# Autodesk Inventor assembly: Frame
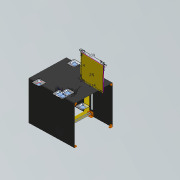
[picture p0: Inventor's stored thumbnail of the model, 180x180]
Saved by Autodesk Inventor 2016 (Build 200138000, 138)
## iProperties
Created: 2016-08-20
Part Number: Frame
Document SubType Name: Assembly
Designer: Sam
Author: Sam
## Documents named in this file (22)
- D:\Users\Sam\Documents\Inventor\Zircon3D\Frame.iam
- D:\Users\Sam\Documents\Inventor\Zircon3D\FrameBase.ipt
- D:\Users\Sam\Documents\Inventor\Zircon3D\FrameCentre.ipt
- D:\Users\Sam\Documents\Inventor\Zircon3D\FrameBack.ipt
- D:\Users\Sam\Documents\Inventor\Zircon3D\Frame3WayBlock.ipt
- D:\Users\Sam\Documents\Inventor\Zircon3D\FrameLeftSide.ipt
- D:\Users\Sam\Documents\Inventor\Zircon3D\FrameTop.ipt
- D:\Users\Sam\Documents\Inventor\Zircon3D\Frame2WayBlock.ipt
- D:\Users\Sam\Documents\Inventor\Zircon3D\FrameRightSide.ipt
- D:\Users\Sam\Documents\Inventor\Zircon3D\Frame Front.ipt
- D:\Users\Sam\Documents\Inventor\Zircon3D\Frame3WayBlockMotor.ipt
- D:\Users\Sam\Documents\Inventor\Zircon3D\SmoothRods.ipt
- D:\Users\Sam\Documents\Inventor\Zircon3D\MotorMountRight.ipt
- D:\Users\Sam\Documents\Inventor\Zircon3D\Frame3WayBlockMotor_MIR.ipt
- D:\Users\Sam\Documents\Inventor\Zircon3D\Nema17.ipt
- D:\Users\Sam\Documents\Inventor\Zircon3D\shaft couple_flex.ipt
- D:\Users\Sam\Documents\Inventor\Zircon3D\ThreadedRod.ipt
- D:\Users\Sam\Documents\Inventor\Zircon3D\YCarriage.ipt
- D:\Users\Sam\Documents\Inventor\Zircon3D\HeatedBed.ipt
- D:\Users\Sam\Documents\Inventor\Zircon3D\MotorMountLeft.ipt
- D:\Users\Sam\Documents\Inventor\Zircon3D\MotorMountLeft_MIR.ipt
- D:\Users\Sam\Documents\Inventor\Zircon3D\XMountL.ipt
## Components (36 placed, 21 different names)
1. FrameBase:1 — Rotational:4, Rotational:5, Rotational:25
2. FrameCentre:1 — Rotational:13, Rotational:15, Rotational:19, Rotational:28, Rotational:29
3. FrameBack:1 — Rotational:3, Rotational:6, Rotational:7, Rotational:10
4. Frame3WayBlock:1 — Rotational:5, Rotational:6
5. Frame3WayBlock:2 — Rotational:3, Rotational:4, Mate:1
6. FrameLeftSide:1 — Mate:1, Rotational:8, Rotational:18, Rotational:24, Rotational:32, Rotational:33
7. FrameTop:1 — Rotational:9, Rotational:11, Rotational:12, Rotational:14, Rotational:22, Rotational:23, Rotational:27
8. Frame3WayBlock:3 — Rotational:7, Rotational:8, Rotational:9
9. Frame3WayBlock:4 — Rotational:12, Rotational:13
10. Frame3WayBlock:5 — Rotational:10, Rotational:11, Rotational:26
11. Frame3WayBlock:6 — Rotational:14, Rotational:15
12. Frame3WayBlock:7 — Rotational:18
13. Frame3WayBlock:8 — Rotational:19
14. Frame2WayBlock:1 — Rotational:22
15. Frame2WayBlock:2 — Rotational:24
16. Frame2WayBlock:3 — Rotational:23
17. Frame2WayBlock:4 — Rotational:25
18. FrameRightSide:1 — Rotational:26
19. Frame Front:1
20. Frame3WayBlockMotor:1 — Rotational:27
21. SmoothRods:1
22. SmoothRods:2 — Mate:3
23. MotorMountRight:1 — Rotational:28, Mate:3, Rotational:31
24. Frame3WayBlockMotor_MIR:1 — Rotational:29
25. Nema17:1 — Cylindrical:2, Rotational:34
26. Nema17:2 — Rotational:31, Cylindrical:1
27. shaft couple_flex:1 — Cylindrical:1, Cylindrical:4
28. shaft couple_flex:2 — Cylindrical:2, Cylindrical:3
29. ThreadedRod:1 — Cylindrical:3
30. ThreadedRod:2 — Cylindrical:4
31. YCarriage:1 — Rigid:1
32. HeatedBed:1 — Rigid:1
33. MotorMountLeft:1 — Rotational:32, Rotational:33, Rotational:34
34. MotorMountLeft_MIR:1
35. XMountL:1 — Rotational:35
36. Nema17:3 — Rotational:35
## Relationships (35: RevoluteJoint 28, CylindricalJoint 4, Mate 2, WeldJoint 1)
- Rotational:3 [RevoluteJoint]: FrameBack:1 ↔ Frame3WayBlock:2
- Rotational:4 [RevoluteJoint]: FrameBase:1 ↔ Frame3WayBlock:2
- Rotational:5 [RevoluteJoint]: FrameBase:1 ↔ Frame3WayBlock:1
- Rotational:6 [RevoluteJoint]: FrameBack:1 ↔ Frame3WayBlock:1
- Mate:1: Frame3WayBlock:2 ↔ FrameLeftSide:1
- Rotational:7 [RevoluteJoint]: FrameBack:1 ↔ Frame3WayBlock:3
- Rotational:8 [RevoluteJoint]: FrameLeftSide:1 ↔ Frame3WayBlock:3
- Rotational:9 [RevoluteJoint]: FrameTop:1 ↔ Frame3WayBlock:3
- Rotational:10 [RevoluteJoint]: FrameBack:1 ↔ Frame3WayBlock:5
- Rotational:11 [RevoluteJoint]: FrameTop:1 ↔ Frame3WayBlock:5
- Rotational:12 [RevoluteJoint]: FrameTop:1 ↔ Frame3WayBlock:4
- Rotational:13 [RevoluteJoint]: FrameCentre:1 ↔ Frame3WayBlock:4
- Rotational:14 [RevoluteJoint]: FrameTop:1 ↔ Frame3WayBlock:6
- Rotational:15 [RevoluteJoint]: FrameCentre:1 ↔ Frame3WayBlock:6
- Rotational:18 [RevoluteJoint]: FrameLeftSide:1 ↔ Frame3WayBlock:7
- Rotational:19 [RevoluteJoint]: FrameCentre:1 ↔ Frame3WayBlock:8
- Rotational:22 [RevoluteJoint]: FrameTop:1 ↔ Frame2WayBlock:1
- Rotational:23 [RevoluteJoint]: FrameTop:1 ↔ Frame2WayBlock:3
- Rotational:24 [RevoluteJoint]: FrameLeftSide:1 ↔ Frame2WayBlock:2
- Rotational:25 [RevoluteJoint]: FrameBase:1 ↔ Frame2WayBlock:4
- Rotational:26 [RevoluteJoint]: Frame3WayBlock:5 ↔ FrameRightSide:1
- Rotational:27 [RevoluteJoint]: FrameTop:1 ↔ Frame3WayBlockMotor:1
- Rotational:28 [RevoluteJoint]: FrameCentre:1 ↔ MotorMountRight:1
- Mate:3: SmoothRods:2 ↔ MotorMountRight:1
- Rotational:29 [RevoluteJoint]: FrameCentre:1 ↔ Frame3WayBlockMotor_MIR:1
- Rotational:31 [RevoluteJoint]: MotorMountRight:1 ↔ Nema17:2
- Cylindrical:1: Nema17:2 ↔ shaft couple_flex:1
- Cylindrical:2: Nema17:1 ↔ shaft couple_flex:2
- Cylindrical:3: shaft couple_flex:2 ↔ ThreadedRod:1
- Cylindrical:4: shaft couple_flex:1 ↔ ThreadedRod:2
- Rigid:1 [WeldJoint] (2.4 mm): YCarriage:1 ↔ HeatedBed:1
- Rotational:32 [RevoluteJoint]: FrameLeftSide:1 ↔ MotorMountLeft:1
- Rotational:33 [RevoluteJoint]: FrameLeftSide:1 ↔ MotorMountLeft:1
- Rotational:34 [RevoluteJoint]: Nema17:1 ↔ MotorMountLeft:1
- Rotational:35 [RevoluteJoint]: XMountL:1 ↔ Nema17:3
